# Autodesk Inventor assembly: C4
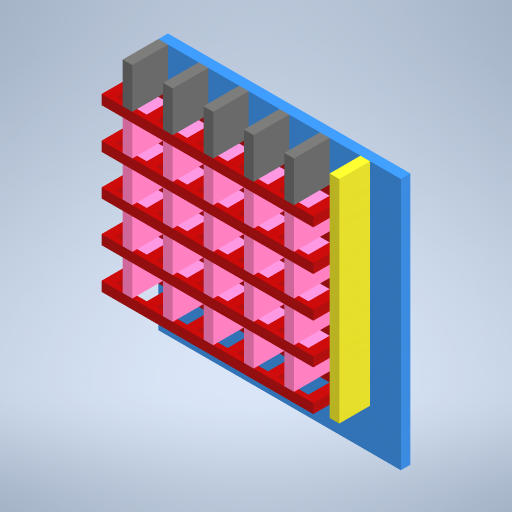
[picture p0: Inventor's stored thumbnail of the model, 512x512]
Saved by Autodesk Inventor 2024 (Build 280153000, 153)
## iProperties
Created: 2023-10-03
Part Number: C4
Document SubType Name: Assembly
Designer: flynf
Author: flynf
## Documents named in this file (6)
- C:\Users\flynf\Documents\C4.iam
- C:\Users\flynf\Documents\FrntBck Plate.ipt
- C:\Users\flynf\Documents\Spacer Bg.ipt
- C:\Users\flynf\Documents\Spacer Sm.ipt
- C:\Users\flynf\Documents\Side Plate.ipt
- C:\Users\flynf\Documents\Slide.ipt
## Components (32 placed, 5 different names)
1. FrntBck Plate:1 — Mate:1, Mate:2, Mate:3, Mate:4, Mate:5, Flush:1, Flush:2, Flush:3, Flush:4, Flush:5, Flush:6, Mate:10, Flush:7, Flush:8, Mate:11, Mate:12, Mate:13, Mate:14, Mate:15, Flush:9, Flush:10, Flush:11, Flush:12, Flush:13, Mate:16, Mate:17, Mate:18, Mate:19, Mate:20, Flush:19, Flush:20, Flush:21, Flush:22, Flush:23, Mate:21, Mate:22, Mate:23, Mate:24, Mate:25, Flush:29, Flush:30, Flush:31, Flush:32, Flush:33, Mate:26, Mate:27, Mate:28, Mate:29, Mate:30, Flush:40, Flush:41, Flush:42, Flush:43, Flush:44, Mate:31, Mate:32, Mate:33, Mate:34, Mate:35, Mate:36, Mate:37, Mate:38, Mate:39, Mate:40
2. Spacer Bg:1 — Mate:5, Flush:5, Mate:9, Flush:18
3. Spacer Bg:2 — Mate:4, Flush:4, Mate:8, Mate:9, Flush:17
4. Spacer Bg:3 — Mate:3, Flush:3, Mate:7, Mate:8, Flush:16
5. Spacer Bg:4 — Mate:2, Flush:2, Mate:6, Mate:7, Flush:15
6. Spacer Bg:5 — Mate:1, Flush:1, Flush:6, Mate:6, Flush:14
7. Side Plate:1 — Mate:10, Flush:7, Flush:8, Mate:41, Mate:42, Mate:43, Mate:44, Mate:45
8. Spacer Sm:1 — Mate:22, Flush:32, Flush:35, Flush:46
9. Spacer Sm:2 — Mate:21, Flush:33, Flush:34, Flush:45
10. Spacer Sm:3 — Mate:13, Flush:11, Flush:16, Flush:26
11. Spacer Sm:4 — Mate:19, Flush:22, Flush:27, Flush:37, Flush:38
12. Spacer Sm:5 — Mate:20, Flush:23, Flush:28, Flush:39
13. Spacer Sm:6 — Mate:15, Flush:9, Flush:18, Flush:28
14. Spacer Sm:7 — Mate:16, Flush:19, Flush:24, Flush:34
15. Spacer Sm:8 — Mate:14, Flush:10, Flush:17, Flush:27
16. Spacer Sm:9 — Mate:12, Flush:12, Flush:15, Flush:25
17. Spacer Sm:10 — Mate:11, Flush:13, Flush:14, Flush:24
18. Spacer Sm:11 — Mate:24, Flush:30, Flush:37, Flush:38, Flush:48
19. Spacer Sm:12 — Mate:26, Flush:44, Flush:45
20. Spacer Sm:13 — Mate:18, Flush:21, Flush:26, Flush:36
21. Spacer Sm:14 — Mate:17, Flush:20, Flush:25, Flush:35
22. Spacer Sm:15 — Mate:25, Flush:29, Flush:39, Flush:49
23. Spacer Sm:16 — Mate:28, Flush:42, Flush:47
24. Spacer Sm:17 — Mate:27, Flush:43, Flush:46
25. Spacer Sm:18 — Mate:29, Flush:41, Flush:48
26. Spacer Sm:19 — Mate:30, Flush:40, Flush:49
27. Spacer Sm:20 — Mate:23, Flush:31, Flush:36, Flush:47
28. Slide:1 — Mate:31, Mate:36, Mate:45
29. Slide:2 — Mate:32, Mate:37, Mate:44
30. Slide:3 — Mate:33, Mate:38, Mate:43
31. Slide:4 — Mate:34, Mate:39, Mate:42
32. Slide:5 — Mate:35, Mate:40, Mate:41
## Relationships (94: Flush 49, Mate 45)
- Mate:1: FrntBck Plate:1 ↔ Spacer Bg:5
- Mate:2: FrntBck Plate:1 ↔ Spacer Bg:4
- Mate:3: FrntBck Plate:1 ↔ Spacer Bg:3
- Mate:4: FrntBck Plate:1 ↔ Spacer Bg:2
- Mate:5: FrntBck Plate:1 ↔ Spacer Bg:1
- Flush:1: FrntBck Plate:1 ↔ Spacer Bg:5
- Flush:2: FrntBck Plate:1 ↔ Spacer Bg:4
- Flush:3: FrntBck Plate:1 ↔ Spacer Bg:3
- Flush:4: FrntBck Plate:1 ↔ Spacer Bg:2
- Flush:5: FrntBck Plate:1 ↔ Spacer Bg:1
- Flush:6: FrntBck Plate:1 ↔ Spacer Bg:5
- Mate:6 (40.64 mm): Spacer Bg:4 ↔ Spacer Bg:5
- Mate:7 (40.64 mm): Spacer Bg:3 ↔ Spacer Bg:4
- Mate:8 (40.64 mm): Spacer Bg:2 ↔ Spacer Bg:3
- Mate:9 (40.64 mm): Spacer Bg:1 ↔ Spacer Bg:2
- Mate:10: FrntBck Plate:1 ↔ Side Plate:1
- Flush:7: FrntBck Plate:1 ↔ Side Plate:1
- Flush:8: FrntBck Plate:1 ↔ Side Plate:1
- Mate:11: FrntBck Plate:1 ↔ Spacer Sm:10
- Mate:12: FrntBck Plate:1 ↔ Spacer Sm:9
- Mate:13: FrntBck Plate:1 ↔ Spacer Sm:3
- Mate:14: FrntBck Plate:1 ↔ Spacer Sm:8
- Mate:15: FrntBck Plate:1 ↔ Spacer Sm:6
- Flush:9: FrntBck Plate:1 ↔ Spacer Sm:6
- Flush:10: FrntBck Plate:1 ↔ Spacer Sm:8
- Flush:11: FrntBck Plate:1 ↔ Spacer Sm:3
- Flush:12: FrntBck Plate:1 ↔ Spacer Sm:9
- Flush:13: FrntBck Plate:1 ↔ Spacer Sm:10
- Flush:14: Spacer Bg:5 ↔ Spacer Sm:10
- Flush:15: Spacer Bg:4 ↔ Spacer Sm:9
- Flush:16: Spacer Bg:3 ↔ Spacer Sm:3
- Flush:17: Spacer Bg:2 ↔ Spacer Sm:8
- Flush:18: Spacer Bg:1 ↔ Spacer Sm:6
- Mate:16: FrntBck Plate:1 ↔ Spacer Sm:7
- Mate:17: FrntBck Plate:1 ↔ Spacer Sm:14
- Mate:18: FrntBck Plate:1 ↔ Spacer Sm:13
- Mate:19: FrntBck Plate:1 ↔ Spacer Sm:4
- Mate:20: FrntBck Plate:1 ↔ Spacer Sm:5
- Flush:19: FrntBck Plate:1 ↔ Spacer Sm:7
- Flush:20: FrntBck Plate:1 ↔ Spacer Sm:14
- Flush:21: FrntBck Plate:1 ↔ Spacer Sm:13
- Flush:22: FrntBck Plate:1 ↔ Spacer Sm:4
- Flush:23: FrntBck Plate:1 ↔ Spacer Sm:5
- Flush:24: Spacer Sm:7 ↔ Spacer Sm:10
- Flush:25: Spacer Sm:9 ↔ Spacer Sm:14
- Flush:26: Spacer Sm:3 ↔ Spacer Sm:13
- Flush:27: Spacer Sm:4 ↔ Spacer Sm:8
- Flush:28: Spacer Sm:5 ↔ Spacer Sm:6
- Mate:21: FrntBck Plate:1 ↔ Spacer Sm:2
- Mate:22: FrntBck Plate:1 ↔ Spacer Sm:1
- Mate:23: FrntBck Plate:1 ↔ Spacer Sm:20
- Mate:24: FrntBck Plate:1 ↔ Spacer Sm:11
- Mate:25: FrntBck Plate:1 ↔ Spacer Sm:15
- Flush:29: FrntBck Plate:1 ↔ Spacer Sm:15
- Flush:30: FrntBck Plate:1 ↔ Spacer Sm:11
- Flush:31: FrntBck Plate:1 ↔ Spacer Sm:20
- Flush:32: FrntBck Plate:1 ↔ Spacer Sm:1
- Flush:33: FrntBck Plate:1 ↔ Spacer Sm:2
- Flush:34: Spacer Sm:2 ↔ Spacer Sm:7
- Flush:35: Spacer Sm:1 ↔ Spacer Sm:14
- Flush:36: Spacer Sm:13 ↔ Spacer Sm:20
- Flush:37: Spacer Sm:4 ↔ Spacer Sm:11
- Flush:38: Spacer Sm:4 ↔ Spacer Sm:11
- Flush:39: Spacer Sm:5 ↔ Spacer Sm:15
- Mate:26: FrntBck Plate:1 ↔ Spacer Sm:12
- Mate:27: FrntBck Plate:1 ↔ Spacer Sm:17
- Mate:28: FrntBck Plate:1 ↔ Spacer Sm:16
- Mate:29: FrntBck Plate:1 ↔ Spacer Sm:18
- Mate:30: FrntBck Plate:1 ↔ Spacer Sm:19
- Flush:40: FrntBck Plate:1 ↔ Spacer Sm:19
- Flush:41: FrntBck Plate:1 ↔ Spacer Sm:18
- Flush:42: FrntBck Plate:1 ↔ Spacer Sm:16
- Flush:43: FrntBck Plate:1 ↔ Spacer Sm:17
- Flush:44: FrntBck Plate:1 ↔ Spacer Sm:12
- Flush:45: Spacer Sm:2 ↔ Spacer Sm:12
- Flush:46: Spacer Sm:1 ↔ Spacer Sm:17
- Flush:47: Spacer Sm:16 ↔ Spacer Sm:20
- Flush:48: Spacer Sm:11 ↔ Spacer Sm:18
- Flush:49: Spacer Sm:15 ↔ Spacer Sm:19
- Mate:31: FrntBck Plate:1 ↔ Slide:1
- Mate:32: FrntBck Plate:1 ↔ Slide:2
- Mate:33: FrntBck Plate:1 ↔ Slide:3
- Mate:34: FrntBck Plate:1 ↔ Slide:4
- Mate:35: FrntBck Plate:1 ↔ Slide:5
- Mate:36: FrntBck Plate:1 ↔ Slide:1
- Mate:37: FrntBck Plate:1 ↔ Slide:2
- Mate:38: FrntBck Plate:1 ↔ Slide:3
- Mate:39: FrntBck Plate:1 ↔ Slide:4
- Mate:40: FrntBck Plate:1 ↔ Slide:5
- Mate:41 (15.24 mm): Side Plate:1 ↔ Slide:5
- Mate:42 (15.24 mm): Side Plate:1 ↔ Slide:4
- Mate:43 (15.24 mm): Side Plate:1 ↔ Slide:3
- Mate:44 (15.24 mm): Side Plate:1 ↔ Slide:2
- Mate:45 (15.24 mm): Side Plate:1 ↔ Slide:1
